# Autodesk Inventor assembly: extension arm spool assembly
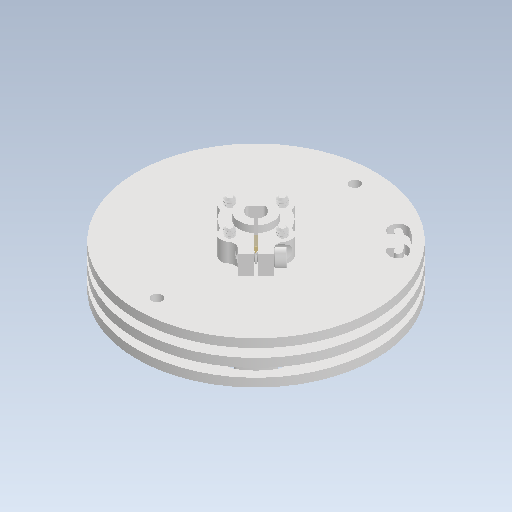
[picture p0: Inventor's stored thumbnail of the model, 512x512]
Saved by Autodesk Inventor 2020 (Build 240168000, 168)
## iProperties
Created: 2020-01-05
Part Number: extension arm spool assembly
Document SubType Name: Assembly
Designer: ball
Author: ball
## Documents named in this file (4)
- D:\FTC8863\2019 Robot\Delivery\extension arm\extension arm spool assembly.iam
- D:\FTC8863\2019 Robot\Delivery\extension arm\extension arm spool 2_75.iam
- D:\FTC8863\Actobotics\545 parts\545619 assembly.ipt
- D:\FTC8863\StepLibraries\Screws\6-32 x 1.000 SOCKET HEAD CAP SCREW.ipt
## Components (6 placed, 3 different names)
1. extension arm spool 2_75:1 [sub-assembly] — Mate:4, Mate:5, Mate:6, Mate:7, Mate:8, Mate:9, Mate:10, Mate:11, Mate:12
2. 6-32 x 1.000 SOCKET HEAD CAP SCREW:1 — Mate:4, Mate:5, Mate:13
3. 6-32 x 1.000 SOCKET HEAD CAP SCREW:2 — Mate:10, Mate:11
4. 6-32 x 1.000 SOCKET HEAD CAP SCREW:3 — Mate:8, Mate:9, Mate:14
5. 6-32 x 1.000 SOCKET HEAD CAP SCREW:4 — Mate:6, Mate:7
6. 545619 assembly:2 — Mate:12, Mate:13, Mate:14
## Relationships (11: Mate 11)
- Mate:4: extension arm spool 2_75:1 ↔ 6-32 x 1.000 SOCKET HEAD CAP SCREW:1
- Mate:5: extension arm spool 2_75:1 ↔ 6-32 x 1.000 SOCKET HEAD CAP SCREW:1
- Mate:6: extension arm spool 2_75:1 ↔ 6-32 x 1.000 SOCKET HEAD CAP SCREW:4
- Mate:7: extension arm spool 2_75:1 ↔ 6-32 x 1.000 SOCKET HEAD CAP SCREW:4
- Mate:8: extension arm spool 2_75:1 ↔ 6-32 x 1.000 SOCKET HEAD CAP SCREW:3
- Mate:9: extension arm spool 2_75:1 ↔ 6-32 x 1.000 SOCKET HEAD CAP SCREW:3
- Mate:10: extension arm spool 2_75:1 ↔ 6-32 x 1.000 SOCKET HEAD CAP SCREW:2
- Mate:11: extension arm spool 2_75:1 ↔ 6-32 x 1.000 SOCKET HEAD CAP SCREW:2
- Mate:12: extension arm spool 2_75:1 ↔ 545619 assembly:2
- Mate:13: 6-32 x 1.000 SOCKET HEAD CAP SCREW:1 ↔ 545619 assembly:2
- Mate:14: 6-32 x 1.000 SOCKET HEAD CAP SCREW:3 ↔ 545619 assembly:2
